# Autodesk Inventor assembly: Section_Pump_Assembly
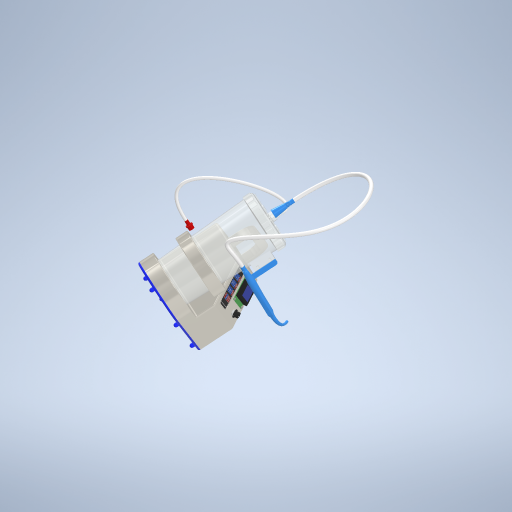
[picture p0: Inventor's stored thumbnail of the model, 512x512]
Saved by Autodesk Inventor 2024 (Build 280153000, 153)
## iProperties
Created: 2024-05-20
Part Number: Section_Pump_Assembly
Document SubType Name: Assembly
Designer: ASUS
Author: ASUS
## Documents named in this file (18)
- C:\Users\ASUS\Documents\Inventor\Tugas Akhir Stechoq\Assembly\Suction_Pump_Assembly.iam
- C:\Users\ASUS\Documents\Inventor\Tugas Akhir Stechoq\Part\Handle_Part.ipt
- C:\Users\ASUS\Documents\Inventor\Tugas Akhir Stechoq\Part\Keypad 4x4.ipt
- C:\Users\ASUS\Documents\Inventor\Tugas Akhir Stechoq\Part\Main_Cover.ipt
- C:\Users\ASUS\Documents\Inventor\Tugas Akhir Stechoq\Part\ScrewM3x0.5_Buttom_Cover.ipt
- C:\Users\ASUS\Documents\Inventor\Tugas Akhir Stechoq\Part\ScrewM3.5x0.6_LCD_Part.ipt
- C:\Users\ASUS\Downloads\rv24yn-1.snapshot.5\RV24 v6\Body v5.ipt
- C:\Users\ASUS\Downloads\rv24yn-1.snapshot.5\RV24 v6\Engraver v3.ipt
- C:\Users\ASUS\Downloads\rv24yn-1.snapshot.5\RV24 v6\Nut M9 v2.ipt
- C:\Users\ASUS\Downloads\rv24yn-1.snapshot.5\RV24 v6\Puck M9 v2.ipt
- C:\Users\ASUS\Downloads\rv24yn-1.snapshot.5\RV24 v6\Shaft v3.ipt
- C:\Users\ASUS\Documents\Inventor\Tugas Akhir Stechoq\Part\ScrewM5x0.8_Handle.ipt
- C:\Users\ASUS\Documents\Inventor\Tugas Akhir Stechoq\Desain Botol\boto suction pump.iam
- C:\Users\ASUS\Documents\Inventor\Tugas Akhir Stechoq\Assembly\Buttom Cover PCB.iam
- Assembly_Buttom_Cover.iam
- C:\Users\ASUS\Documents\Inventor\Tugas Akhir Stechoq\Part\power connector.ipt
- C:\Users\ASUS\Documents\Inventor\Tugas Akhir Stechoq\Assembly\Lcd i2c.iam
- C:\Users\ASUS\Documents\Inventor\Tugas Akhir Stechoq\Part\Potentiometer Knob.ipt
## Components (25 placed, 16 different names)
1. Handle_Part:1 — Transitional:1, Mate:35, Mate:74, Mate:75, Mate:76, Mate:77, Mate:78
2. Keypad 4x4:1 — Mate:4, Mate:5, Mate:6
3. Main_Cover:1 — Mate:4, Mate:5, Mate:6, Transitional:1, Mate:35, Mate:43, Mate:44, Mate:72, Mate:73, Mate:76, Mate:77, Mate:78, Mate:96, Mate:97, Mate:98, Mate:101, Mate:105, Mate:106, Mate:107, Mate:108, Mate:118, Mate:119, Mate:120, Mate:121, Mate:122, Mate:123
4. ScrewM3x0.5_Buttom_Cover:2 — Mate:126, Mate:127
5. ScrewM3x0.5_Buttom_Cover:3 — Mate:124, Mate:125
6. ScrewM3x0.5_Buttom_Cover:4 — Mate:128, Mate:129
7. ScrewM3.5x0.6_LCD_Part:1 — Mate:111, Mate:112
8. ScrewM3.5x0.6_LCD_Part:2 — Mate:117, Mate:118
9. ScrewM3.5x0.6_LCD_Part:3 — Mate:115, Mate:116
10. ScrewM3.5x0.6_LCD_Part:4 — Mate:113, Mate:114
11. Body v5:1 — Mate:41, Mate:42, Mate:43, Mate:45, Mate:57, Mate:58, Mate:108, Mate:109
12. Engraver v3:1 — Mate:39, Mate:40, Mate:42, Mate:110
13. Nut M9 v2:1 — Mate:44, Mate:45, Mate:109, Mate:110
14. Puck M9 v2:1 — Mate:39, Mate:40, Mate:41
15. Shaft v3:1 — Mate:57, Mate:58, Mate:132, Mate:133
16. ScrewM5x0.8_Handle:1 — Mate:72, Mate:74
17. ScrewM5x0.8_Handle:2 — Mate:73, Mate:75
18. boto suction pump:1 [sub-assembly] — Mate:119, Mate:120
19. power connector:1 — Mate:96, Mate:97, Mate:98, Mate:99, Mate:100, Mate:102
20. ScrewM3.5x0.6_LCD_Part:5 — Mate:99, Mate:100
21. ScrewM3.5x0.6_LCD_Part:6 — Mate:101, Mate:102
22. Lcd i2c:1 [sub-assembly] — Mate:105, Mate:106, Mate:107, Mate:111, Mate:112, Mate:113, Mate:114, Mate:115, Mate:116, Mate:117
23. Assembly_Buttom_Cover:1 [sub-assembly] — Mate:121, Mate:122, Mate:123, Mate:124, Mate:125, Mate:126, Mate:127, Mate:128, Mate:129, Mate:130, Mate:131
24. ScrewM3x0.5_Buttom_Cover:5 — Mate:130, Mate:131
25. Potentiometer Knob:1 — Mate:132, Mate:133
## Relationships (57: Mate 56, Transitional 1)
- Mate:4: Keypad 4x4:1 ↔ Main_Cover:1
- Mate:5: Keypad 4x4:1 ↔ Main_Cover:1
- Mate:6: Keypad 4x4:1 ↔ Main_Cover:1
- Transitional:1: Handle_Part:1 ↔ Main_Cover:1
- Mate:35: Handle_Part:1 ↔ Main_Cover:1
- Mate:39: Engraver v3:1 ↔ Puck M9 v2:1
- Mate:40: Engraver v3:1 ↔ Puck M9 v2:1
- Mate:41: Body v5:1 ↔ Puck M9 v2:1
- Mate:42: Body v5:1 ↔ Engraver v3:1
- Mate:43: Main_Cover:1 ↔ Body v5:1
- Mate:44: Main_Cover:1 ↔ Nut M9 v2:1
- Mate:45: Body v5:1 ↔ Nut M9 v2:1
- Mate:57: Body v5:1 ↔ Shaft v3:1
- Mate:58: Body v5:1 ↔ Shaft v3:1
- Mate:72: Main_Cover:1 ↔ ScrewM5x0.8_Handle:1
- Mate:73: Main_Cover:1 ↔ ScrewM5x0.8_Handle:2
- Mate:74: Handle_Part:1 ↔ ScrewM5x0.8_Handle:1
- Mate:75: Handle_Part:1 ↔ ScrewM5x0.8_Handle:2
- Mate:76: Handle_Part:1 ↔ Main_Cover:1
- Mate:77: Handle_Part:1 ↔ Main_Cover:1
- Mate:78: Handle_Part:1 ↔ Main_Cover:1
- Mate:96: Main_Cover:1 ↔ power connector:1
- Mate:97: Main_Cover:1 ↔ power connector:1
- Mate:98: Main_Cover:1 ↔ power connector:1
- Mate:99: power connector:1 ↔ ScrewM3.5x0.6_LCD_Part:5
- Mate:100: power connector:1 ↔ ScrewM3.5x0.6_LCD_Part:5
- Mate:101: Main_Cover:1 ↔ ScrewM3.5x0.6_LCD_Part:6
- Mate:102: power connector:1 ↔ ScrewM3.5x0.6_LCD_Part:6
- Mate:105: Main_Cover:1 ↔ Lcd i2c:1
- Mate:106: Main_Cover:1 ↔ Lcd i2c:1
- Mate:107: Main_Cover:1 ↔ Lcd i2c:1
- Mate:108: Main_Cover:1 ↔ Body v5:1
- Mate:109: Body v5:1 ↔ Nut M9 v2:1
- Mate:110 (-5 mm): Engraver v3:1 ↔ Nut M9 v2:1
- Mate:111: ScrewM3.5x0.6_LCD_Part:1 ↔ Lcd i2c:1
- Mate:112: ScrewM3.5x0.6_LCD_Part:1 ↔ Lcd i2c:1
- Mate:113: ScrewM3.5x0.6_LCD_Part:4 ↔ Lcd i2c:1
- Mate:114: ScrewM3.5x0.6_LCD_Part:4 ↔ Lcd i2c:1
- Mate:115: ScrewM3.5x0.6_LCD_Part:3 ↔ Lcd i2c:1
- Mate:116: ScrewM3.5x0.6_LCD_Part:3 ↔ Lcd i2c:1
- Mate:117: ScrewM3.5x0.6_LCD_Part:2 ↔ Lcd i2c:1
- Mate:118: Main_Cover:1 ↔ ScrewM3.5x0.6_LCD_Part:2
- Mate:119: Main_Cover:1 ↔ boto suction pump:1
- Mate:120: Main_Cover:1 ↔ boto suction pump:1
- Mate:121: Main_Cover:1 ↔ Assembly_Buttom_Cover:1
- Mate:122: Main_Cover:1 ↔ Assembly_Buttom_Cover:1
- Mate:123: Main_Cover:1 ↔ Assembly_Buttom_Cover:1
- Mate:124: ScrewM3x0.5_Buttom_Cover:3 ↔ Assembly_Buttom_Cover:1
- Mate:125: ScrewM3x0.5_Buttom_Cover:3 ↔ Assembly_Buttom_Cover:1
- Mate:126: ScrewM3x0.5_Buttom_Cover:2 ↔ Assembly_Buttom_Cover:1
- Mate:127: ScrewM3x0.5_Buttom_Cover:2 ↔ Assembly_Buttom_Cover:1
- Mate:128: ScrewM3x0.5_Buttom_Cover:4 ↔ Assembly_Buttom_Cover:1
- Mate:129: ScrewM3x0.5_Buttom_Cover:4 ↔ Assembly_Buttom_Cover:1
- Mate:130: Assembly_Buttom_Cover:1 ↔ ScrewM3x0.5_Buttom_Cover:5
- Mate:131: Assembly_Buttom_Cover:1 ↔ ScrewM3x0.5_Buttom_Cover:5
- Mate:132: Shaft v3:1 ↔ Potentiometer Knob:1
- Mate:133: Shaft v3:1 ↔ Potentiometer Knob:1
